# Autodesk Inventor assembly: RearZMotorMount
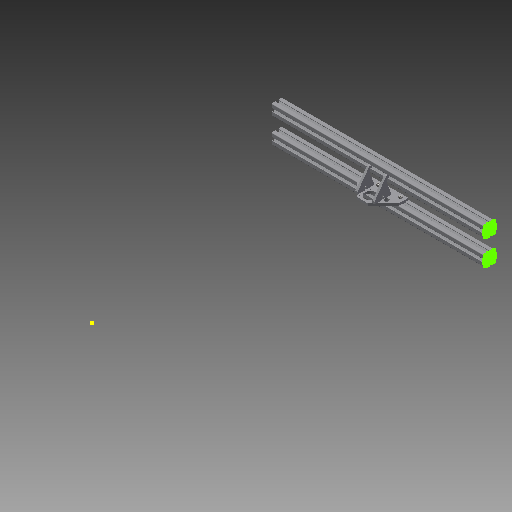
[picture p0: Inventor's stored thumbnail of the model, 512x512]
Saved by Autodesk Inventor 2018 (Build 220112000, 112)
## iProperties
Created: 2016-08-03
Part Number: RearZMotorMount
Document SubType Name: Assembly
Designer: User
Author: User
## Documents named in this file (4)
- C:\Users\Dan\OneDrive\SL-Inventor\The Beast v1.2 PackandGo\Workspaces\Workspace\RearZMotorMount.iam
- C:\Users\Dan\OneDrive\SL-Inventor\The Beast v1.2 PackandGo\Workspaces\Workspace\3030 600mm_CPY.ipt
- C:\Users\Dan\OneDrive\SL-Inventor\The Beast v1.2 PackandGo\Workspaces\Workspace\Z Motor Mount.iam
- C:\Users\Dan\OneDrive\SL-Inventor\The Beast v1.2 PackandGo\Workspaces\Workspace\Lower Panels.iam
## Components (4 placed, 3 different names)
1. 3030 600mm_CPY:1
2. 3030 600mm_CPY:2
3. Z Motor Mount:1 [sub-assembly]
4. Lower Panels:1 [sub-assembly]
## Relationships (3: Flush 1, Angle 1, Mate 1)
- [Flush]: 3030 600mm_CPY:1 ↔ Lower Panels:1
- [Angle] (180 deg): 3030 600mm_CPY:2 ↔ Z Motor Mount:1
- [Mate]: 3030 600mm_CPY:1 ↔ Lower Panels:1
